# Autodesk Inventor assembly: robot
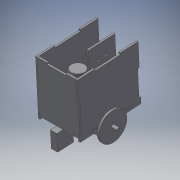
[picture p0: Inventor's stored thumbnail of the model, 180x180]
Saved by Autodesk Inventor 2019 (Build 230136000, 136)
## iProperties
Created: 2018-09-07
Part Number: robot
Document SubType Name: Assembly
Designer: mspet
Author: mspet
## Documents named in this file (10)
- C:\Users\mspet\Desktop\Simon\CAD\robot.iam
- C:\Users\mspet\Desktop\Simon\CAD\side.ipt
- C:\Users\mspet\Desktop\Simon\CAD\motor.ipt
- C:\Users\mspet\Desktop\Simon\CAD\wheel.ipt
- C:\Users\mspet\Desktop\Simon\CAD\base.ipt
- C:\Users\mspet\Desktop\Simon\CAD\caster.ipt
- C:\Users\mspet\Desktop\Simon\CAD\rib.ipt
- C:\Users\mspet\Desktop\Simon\CAD\wheel_acry.ipt
- C:\Users\mspet\Desktop\Simon\CAD\back.ipt
- C:\Users\mspet\Desktop\Simon\CAD\top.ipt
## Components (14 placed, 9 different names)
1. side:1 — Mate:1, Mate:2, Mate:3, Flush:1, Mate:4, Mate:5, Mate:28, Mate:29, Mate:30, Mate:31
2. motor:1 — Mate:1, Mate:2, Mate:24
3. wheel:1 — Mate:3
4. base:1 — Flush:1, Mate:4, Mate:5, Mate:6, Mate:9, Mate:10, Mate:11, Mate:12, Mate:13, Mate:17, Mate:18, Mate:19, Mate:25, Mate:26, Mate:27
5. caster:1 — Mate:6, Mate:10, Mate:11
6. caster:2 — Mate:9, Mate:12, Mate:13
7. side:2 — Mate:17, Mate:18, Mate:19
8. motor:2 — Mate:23
9. wheel:2
10. rib:1 — Mate:25, Mate:26, Mate:27
11. wheel_acry:1 — Mate:23
12. wheel_acry:2 — Mate:24
13. back:1 — Mate:28, Mate:29, Mate:30, Flush:2, Mate:32
14. top:1 — Mate:31, Flush:2, Mate:32
## Relationships (29: Mate 27, Flush 2)
- Mate:1: side:1 ↔ motor:1
- Mate:2: side:1 ↔ motor:1
- Mate:3: side:1 ↔ wheel:1
- Flush:1: side:1 ↔ base:1
- Mate:4: side:1 ↔ base:1
- Mate:5: side:1 ↔ base:1
- Mate:6: base:1 ↔ caster:1
- Mate:9: base:1 ↔ caster:2
- Mate:10: base:1 ↔ caster:1
- Mate:11: base:1 ↔ caster:1
- Mate:12: base:1 ↔ caster:2
- Mate:13: base:1 ↔ caster:2
- [Mate]: side:2 ↔ motor:2
- [Mate]: side:2 ↔ motor:2
- [Mate]: side:2 ↔ wheel:2
- Mate:17: base:1 ↔ side:2
- Mate:18: base:1 ↔ side:2
- Mate:19: base:1 ↔ side:2
- Mate:23: motor:2 ↔ wheel_acry:1
- Mate:24: motor:1 ↔ wheel_acry:2
- Mate:25: base:1 ↔ rib:1
- Mate:26: base:1 ↔ rib:1
- Mate:27: base:1 ↔ rib:1
- Mate:28: side:1 ↔ back:1
- Mate:29: side:1 ↔ back:1
- Mate:30: side:1 ↔ back:1
- Mate:31: side:1 ↔ top:1
- Flush:2: back:1 ↔ top:1
- Mate:32: back:1 ↔ top:1
## Named parameters: d20_d3 = 0 mm, d21_d0 = 0 mm, d22_d1 = 0 mm
